# Autodesk Inventor assembly: cRIO with Modules
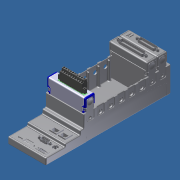
[picture p0: Inventor's stored thumbnail of the model, 180x180]
Saved by Autodesk Inventor 2012 (Build 160160000, 160)
## iProperties
Created: 2012-03-15
Part Number: cRIO with Modules
Document SubType Name: Assembly
Designer: Ed
Author: Ed
## Documents named in this file (6)
- C:\Users\Ed\Documents\masters\CAD\cRIO\Inventor\cRIO with Modules.iam
- C:\Users\Ed\Documents\masters\CAD\cRIO\Inventor\crio 9074.ipt
- C:\Users\Ed\Documents\masters\CAD\Imported Components\cu_conn_crio_10_pos_weid\cu_conn_crio_10_pos_weid.ipt
- C:\Users\Ed\Documents\masters\CAD\Imported Components\cu_mod_crio_10_pos_cmbcn\cu_mod_crio_10_pos_cmbcn.ipt
- C:\Users\Ed\Documents\masters\CAD\Imported Components\cu_mod_crio_db_25\cu_mod_crio_db_25.ipt
- C:\Users\Ed\Documents\masters\CAD\Imported Components\cu_mod_crio_db_37\cu_mod_crio_db_37.ipt
## Components (5 placed, 5 different names)
1. crio 9074:1 — Mate:1, Mate:2, Mate:3, Mate:4
2. cu_conn_crio_10_pos_weid:1 — Insert:1, Insert:2
3. cu_mod_crio_10_pos_cmbcn:1 — Flush:5, Flush:6, Insert:1, Insert:2, Mate:4
4. cu_mod_crio_db_25:1 — Mate:1, Flush:3, Flush:4, Mate:2
5. cu_mod_crio_db_37:1 — Flush:3, Flush:4, Flush:5, Flush:6, Mate:3
## Relationships (10: Mate 4, Flush 4, Insert 2)
- Mate:1: crio 9074:1 ↔ cu_mod_crio_db_25:1
- Flush:3: cu_mod_crio_db_25:1 ↔ cu_mod_crio_db_37:1
- Flush:4: cu_mod_crio_db_25:1 ↔ cu_mod_crio_db_37:1
- Flush:5: cu_mod_crio_10_pos_cmbcn:1 ↔ cu_mod_crio_db_37:1
- Flush:6: cu_mod_crio_10_pos_cmbcn:1 ↔ cu_mod_crio_db_37:1
- Insert:1: cu_conn_crio_10_pos_weid:1 ↔ cu_mod_crio_10_pos_cmbcn:1
- Insert:2: cu_conn_crio_10_pos_weid:1 ↔ cu_mod_crio_10_pos_cmbcn:1
- Mate:2: crio 9074:1 ↔ cu_mod_crio_db_25:1
- Mate:3: crio 9074:1 ↔ cu_mod_crio_db_37:1
- Mate:4: crio 9074:1 ↔ cu_mod_crio_10_pos_cmbcn:1
